# Autodesk Inventor assembly: main_assembly
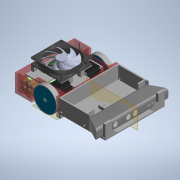
[picture p0: Inventor's stored thumbnail of the model, 180x180]
Saved by Autodesk Inventor 2020 (Build 240168000, 168)
## iProperties
Part Number: main_assembly
Document SubType Name: Assembly
Designer: Abhinav Roy
Author: Abhinav Roy
## Documents named in this file (3)
- D:\Mopping_Robot\cad\V1.0\stl_files\main_assembly.iam
- D:\Mopping_Robot\cad\V1.0\front_assembly.iam
- D:\Mopping_Robot\cad\V1.0\Rear_assembly.iam
## Components (2 placed, 2 different names)
1. front_assembly:1 [sub-assembly] — Mate:1, Mate:2, Mate:3
2. Rear_assembly:1 [sub-assembly] — Mate:1, Mate:2, Mate:3
## Relationships (3: Mate 3)
- Mate:1: front_assembly:1 ↔ Rear_assembly:1
- Mate:2: front_assembly:1 ↔ Rear_assembly:1
- Mate:3: front_assembly:1 ↔ Rear_assembly:1
